# Autodesk Inventor assembly: HbHand
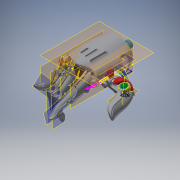
[picture p0: Inventor's stored thumbnail of the model, 180x180]
Saved by Autodesk Inventor 2017 (Build 210142000, 142)
## iProperties
Part Number: HbHand
Material: 一般
Document SubType Name: Assembly
Designer: sktom
Author: sktom
## Documents named in this file (20)
- D:\OneDrive\CAD\MAJ\hackberry\HACKberry-hardware\3D_69%\Inventor\HbHandForChild\HbHand.iam
- D:\OneDrive\CAD\MAJ\hackberry\HACKberry-hardware\3D_69%\Inventor\HbHandForChild\HbPalmBase03ForChild.ipt
- D:\OneDrive\CAD\MAJ\hackberry\HACKberry-hardware\3D_69%\Inventor\HbHandForChild\HbWristMount01ForChild.ipt
- D:\OneDrive\CAD\MAJ\hackberry\HACKberry-hardware\3D_69%\Inventor\HbHandForChild\HbthumbU02ForChild\HbthumbU02ForChild.iam
- D:\OneDrive\CAD\MAJ\hackberry\HACKberry-hardware\3D_69%\Inventor\HbHandForChild\HbFinger01ForChild\HbFinger01ForChild.iam
- D:\OneDrive\CAD\MAJ\hackberry\HACKberry-hardware\3D_69%\Inventor\HbHandForChild\HbShaftStopperB04ForChild.ipt
- D:\OneDrive\CAD\MAJ\hackberry\HACKberry-hardware\3D_69%\Inventor\HbHandForChild\HbFingerMainCouplerLink01ForChild.ipt
- D:\OneDrive\CAD\MAJ\hackberry\HACKberry-hardware\3D_69%\Inventor\HbHandForChild\DummyMetalCollarPh3L5.ipt
- D:\OneDrive\CAD\MAJ\hackberry\HACKberry-hardware\3D_69%\Inventor\HbHandForChild\HbMiddle-RingCouplerLink01ForChild.ipt
- D:\OneDrive\CAD\MAJ\hackberry\HACKberry-hardware\3D_69%\Inventor\HbHandForChild\HbRing-LittleCouplerLink01ForChild.ipt
- D:\OneDrive\CAD\MAJ\hackberry\HACKberry-hardware\3D_69%\Inventor\HbHandForChild\HbIndexFinger01ForChild\HbIndexFinger01ForChild.iam
- D:\OneDrive\CAD\MAJ\hackberry\HACKberry-hardware\3D_69%\Inventor\HbHandForChild\HbShaftStopperA04ForChild.ipt
- D:\OneDrive\CAD\MAJ\hackberry\HACKberry-hardware\3D_69%\Inventor\HbHandForChild\DummyHbServoHorn01.ipt
- D:\OneDrive\CAD\MAJ\hackberry\HACKberry-hardware\3D_69%\Inventor\HbHandForChild\HbIndexMotorGear02ForChild.ipt
- D:\OneDrive\CAD\MAJ\hackberry\HACKberry-hardware\3D_69%\Inventor\HbHandForChild\HbBackCover02ForChild.ipt
- D:\OneDrive\CAD\MAJ\hackberry\HACKberry-hardware\3D_69%\Inventor\HbHandForChild\HbHandBoardMk2_02-3\HbHandBoardMk2_02_12721.iam
- D:\OneDrive\CAD\MAJ\hackberry\HACKberry-hardware\3D_69%\Inventor\HbHandForChild\HbServoHK282A\Servo_HK282A_Hone.ipt
- D:\OneDrive\CAD\MAJ\hackberry\HACKberry-hardware\3D_69%\Inventor\HbHandForChild\HbServoHK282A\Servo_HK282A.ipt
- D:\OneDrive\CAD\MAJ\hackberry\HACKberry-hardware\3D_69%\Inventor\HbHandForChild\bearing_f684zz.ipt
- D:\OneDrive\CAD\MAJ\hackberry\HACKberry-hardware\3D_69%\Inventor\HbHandForChild\servo\GWS_Micro2BBMG.ipt
## Components (27 placed, 19 different names)
1. HbPalmBase03ForChild:1 — 挿入:1, 挿入:2, 挿入:7, 円柱状:1, 挿入:8, 円柱状:2, 挿入:9, 円柱状:3, 挿入:10, 挿入:21, 挿入:22, 挿入:33, 挿入:34, 挿入:36, 挿入:37, 挿入:42, 挿入:43, 挿入:44, 挿入:57
2. HbWristMount01ForChild:1 — 挿入:1, 挿入:2
3. HbthumbU02ForChild:1 [sub-assembly] — 挿入:40, 挿入:41
4. HbFinger01ForChild:1 [sub-assembly] — 挿入:7, 円柱状:1, 挿入:13, 円柱状:5
5. HbFinger01ForChild:2 [sub-assembly] — 挿入:8, 円柱状:2, 挿入:18, 挿入:20
6. HbFinger01ForChild:3 [sub-assembly] — 挿入:9, 円柱状:3, 円柱状:4
7. HbShaftStopperB04ForChild:1 — 挿入:10
8. HbFingerMainCouplerLink01ForChild:1 — 挿入:53, 挿入:56
9. DummyMetalCollarPh3L5:1 — 挿入:13, 挿入:53
10. DummyMetalCollarPh3L5:2 — 挿入:55, 挿入:56
11. DummyMetalCollarPh3L5:3 — 円柱状:5, 挿入:52
12. DummyMetalCollarPh3L5:4 — 挿入:18, 挿入:51
13. DummyMetalCollarPh3L5:5 — 挿入:20, 挿入:50
14. DummyMetalCollarPh3L5:6 — 円柱状:4, 挿入:49
15. HbMiddle-RingCouplerLink01ForChild:1 — 挿入:49, 挿入:50
16. HbRing-LittleCouplerLink01ForChild:1 — 挿入:51, 挿入:52
17. HbIndexFinger01ForChild:1 [sub-assembly] — 挿入:21
18. HbShaftStopperA04ForChild:1 — 挿入:22
19. DummyHbServoHorn01:1 — 挿入:23, 挿入:24
20. HbIndexMotorGear02ForChild:1 — 挿入:23, 挿入:24
21. HbBackCover02ForChild:1 — 挿入:33, 挿入:34, フラッシュ:1
22. HbHandBoardMk2_02_12721:1 [sub-assembly] — 挿入:57, フラッシュ:1
23. Servo_HK282A_Hone:1 — 円柱状:6, 挿入:55
24. Servo_HK282A:1 — 挿入:36, 挿入:37, 円柱状:6
25. bearing_f684zz:1 — 挿入:41, 挿入:42
26. Servo_HK282A_Hone:2 — 挿入:40
27. GWS_Micro2BBMG:1 — 挿入:43, 挿入:44
## Relationships (37: Insert 30, CylindricalJoint 6, Flush 1)
- 挿入:1 [Insert]: HbPalmBase03ForChild:1 ↔ HbWristMount01ForChild:1
- 挿入:2 [Insert]: HbPalmBase03ForChild:1 ↔ HbWristMount01ForChild:1
- 挿入:7 [Insert] (0.5 mm): HbPalmBase03ForChild:1 ↔ HbFinger01ForChild:1
- 円柱状:1 [CylindricalJoint]: HbPalmBase03ForChild:1 ↔ HbFinger01ForChild:1
- 挿入:8 [Insert] (0.5 mm): HbPalmBase03ForChild:1 ↔ HbFinger01ForChild:2
- 円柱状:2 [CylindricalJoint]: HbPalmBase03ForChild:1 ↔ HbFinger01ForChild:2
- 挿入:9 [Insert] (0.5 mm): HbPalmBase03ForChild:1 ↔ HbFinger01ForChild:3
- 円柱状:3 [CylindricalJoint]: HbPalmBase03ForChild:1 ↔ HbFinger01ForChild:3
- 挿入:10 [Insert]: HbPalmBase03ForChild:1 ↔ HbShaftStopperB04ForChild:1
- 挿入:13 [Insert]: HbFinger01ForChild:1 ↔ DummyMetalCollarPh3L5:1
- 挿入:18 [Insert]: HbFinger01ForChild:2 ↔ DummyMetalCollarPh3L5:4
- 挿入:20 [Insert]: HbFinger01ForChild:2 ↔ DummyMetalCollarPh3L5:5
- 円柱状:4 [CylindricalJoint]: HbFinger01ForChild:3 ↔ DummyMetalCollarPh3L5:6
- 円柱状:5 [CylindricalJoint]: HbFinger01ForChild:1 ↔ DummyMetalCollarPh3L5:3
- 挿入:21 [Insert] (0.25 mm): HbPalmBase03ForChild:1 ↔ HbIndexFinger01ForChild:1
- 挿入:22 [Insert]: HbPalmBase03ForChild:1 ↔ HbShaftStopperA04ForChild:1
- 挿入:23 [Insert]: DummyHbServoHorn01:1 ↔ HbIndexMotorGear02ForChild:1
- 挿入:24 [Insert]: DummyHbServoHorn01:1 ↔ HbIndexMotorGear02ForChild:1
- 挿入:33 [Insert]: HbPalmBase03ForChild:1 ↔ HbBackCover02ForChild:1
- 挿入:34 [Insert]: HbPalmBase03ForChild:1 ↔ HbBackCover02ForChild:1
- 挿入:36 [Insert]: HbPalmBase03ForChild:1 ↔ Servo_HK282A:1
- 挿入:37 [Insert]: HbPalmBase03ForChild:1 ↔ Servo_HK282A:1
- 円柱状:6 [CylindricalJoint]: Servo_HK282A_Hone:1 ↔ Servo_HK282A:1
- 挿入:40 [Insert]: HbthumbU02ForChild:1 ↔ Servo_HK282A_Hone:2
- 挿入:41 [Insert]: HbthumbU02ForChild:1 ↔ bearing_f684zz:1
- 挿入:42 [Insert]: HbPalmBase03ForChild:1 ↔ bearing_f684zz:1
- 挿入:43 [Insert]: HbPalmBase03ForChild:1 ↔ GWS_Micro2BBMG:1
- 挿入:44 [Insert]: HbPalmBase03ForChild:1 ↔ GWS_Micro2BBMG:1
- 挿入:49 [Insert] (-0.2 mm): DummyMetalCollarPh3L5:6 ↔ HbMiddle-RingCouplerLink01ForChild:1
- 挿入:50 [Insert]: DummyMetalCollarPh3L5:5 ↔ HbMiddle-RingCouplerLink01ForChild:1
- 挿入:51 [Insert]: DummyMetalCollarPh3L5:4 ↔ HbRing-LittleCouplerLink01ForChild:1
- 挿入:52 [Insert]: DummyMetalCollarPh3L5:3 ↔ HbRing-LittleCouplerLink01ForChild:1
- 挿入:53 [Insert] (-0.5 mm): HbFingerMainCouplerLink01ForChild:1 ↔ DummyMetalCollarPh3L5:1
- 挿入:55 [Insert]: DummyMetalCollarPh3L5:2 ↔ Servo_HK282A_Hone:1
- 挿入:56 [Insert] (-0.2 mm): HbFingerMainCouplerLink01ForChild:1 ↔ DummyMetalCollarPh3L5:2
- 挿入:57 [Insert]: HbPalmBase03ForChild:1 ↔ HbHandBoardMk2_02_12721:1
- フラッシュ:1 [Flush]: HbBackCover02ForChild:1 ↔ HbHandBoardMk2_02_12721:1
